# Autodesk Inventor assembly: Servo_Shaft
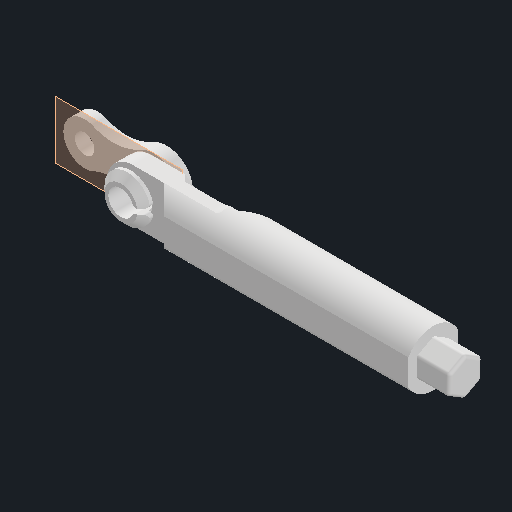
[picture p0: Inventor's stored thumbnail of the model, 512x512]
Saved by Autodesk Inventor 2024 (Build 280153000, 153)
## iProperties
Created: 2025-09-10
Part Number: Servo_Shaft
Document SubType Name: Assembly
Designer: kevin
Author: kevin
## Documents named in this file (3)
- C:\Users\kevin\Desktop\SeniorDesign\Servo_Shaft.iam
- C:\Users\kevin\Desktop\Servo_Pulley.ipt
- C:\Users\kevin\Desktop\SeniorDesign\Shaft_Long.ipt
## Components (2 placed, 2 different names)
1. Servo_Pulley:1 — Flush:1, Flush:2
2. Shaft_Long:1 — Flush:1, Flush:2
## Relationships (2: Flush 2)
- Flush:1: Servo_Pulley:1 ↔ Shaft_Long:1
- Flush:2 (0.762 mm): Servo_Pulley:1 ↔ Shaft_Long:1
